# Autodesk Inventor assembly: Controller
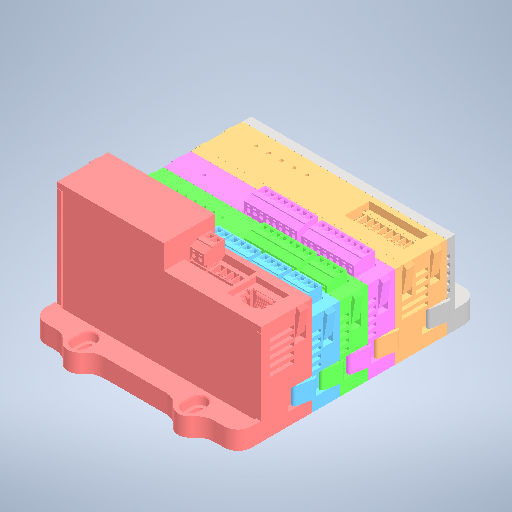
[picture p0: Inventor's stored thumbnail of the model, 512x512]
Saved by Autodesk Inventor 2025.2 (Build 292293000, 293)
## iProperties
Created: 2025-11-01
Part Number: Controller
Document SubType Name: Assembly
Designer: leowa
Author: leowa
## Documents named in this file (8)
- C:\Users\leowa\OneDrive - Fachhochschule Aachen\FH\8. Semester\CANTram-Framework\Inventor CAD\Workspaces\Arbeitsbereich\Module\Controller.iam
- C:\Users\leowa\OneDrive - Fachhochschule Aachen\FH\8. Semester\CANTram-Framework\Inventor CAD\Workspaces\Arbeitsbereich\Module\Analogmodul Baugruppe.iam
- C:\Users\leowa\OneDrive - Fachhochschule Aachen\FH\8. Semester\CANTram-Framework\Inventor CAD\Workspaces\Arbeitsbereich\Module\Busmodul Baugruppe.iam
- C:\Users\leowa\OneDrive - Fachhochschule Aachen\FH\8. Semester\CANTram-Framework\Inventor CAD\Workspaces\Arbeitsbereich\Module\Digitalmodul Baugruppe.iam
- C:\Users\leowa\OneDrive - Fachhochschule Aachen\FH\8. Semester\CANTram-Framework\Inventor CAD\Workspaces\Arbeitsbereich\Module\Hauptmodul.iam
- C:\Users\leowa\OneDrive - Fachhochschule Aachen\FH\8. Semester\CANTram-Framework\Inventor CAD\Workspaces\Arbeitsbereich\Gehäuse\Abschlussmodul.ipt
- C:\Users\leowa\OneDrive - Fachhochschule Aachen\FH\8. Semester\CANTram-Framework\Inventor CAD\Workspaces\Arbeitsbereich\Platinen\Debugmodul\Debugmodul\Debugmodul.iam
- C:\Users\leowa\OneDrive - Fachhochschule Aachen\FH\8. Semester\CANTram-Framework\Inventor CAD\Workspaces\Arbeitsbereich\Module\Relaismodul Baugruppe.iam
## Components (7 placed, 7 different names)
1. Analogmodul Baugruppe:1 [sub-assembly] — Fluchtend:1, Fluchtend:3, Fluchtend:4, Passend:1, Passend:2, Fluchtend:11
2. Busmodul Baugruppe:1 [sub-assembly] — Fluchtend:1, Fluchtend:2, Fluchtend:3, Passend:1, Fluchtend:5, Fluchtend:6, Fluchtend:9, Passend:5, Passend:6, Fluchtend:10, Passend:7
3. Digitalmodul Baugruppe:1 [sub-assembly] — Fluchtend:2, Fluchtend:4, Passend:2, Fluchtend:7, Fluchtend:8, Passend:4
4. Hauptmodul:1 [sub-assembly] — Fluchtend:7, Fluchtend:8, Passend:4
5. Abschlussmodul:1 — Fluchtend:5, Fluchtend:6, Passend:8
6. Debugmodul:1 [sub-assembly] — Fluchtend:9, Passend:5, Passend:6
7. Relaismodul Baugruppe:1 [sub-assembly] — Fluchtend:10, Fluchtend:11, Passend:7, Passend:8
## Relationships (18: Flush 11, Mate 7)
- Fluchtend:1 [Flush]: Analogmodul Baugruppe:1 ↔ Busmodul Baugruppe:1
- Fluchtend:2 [Flush]: Busmodul Baugruppe:1 ↔ Digitalmodul Baugruppe:1
- Fluchtend:3 [Flush]: Analogmodul Baugruppe:1 ↔ Busmodul Baugruppe:1
- Fluchtend:4 [Flush]: Analogmodul Baugruppe:1 ↔ Digitalmodul Baugruppe:1
- Passend:1 [Mate]: Analogmodul Baugruppe:1 ↔ Busmodul Baugruppe:1
- Passend:2 [Mate]: Analogmodul Baugruppe:1 ↔ Digitalmodul Baugruppe:1
- Fluchtend:5 [Flush]: Busmodul Baugruppe:1 ↔ Abschlussmodul:1
- Fluchtend:6 [Flush]: Busmodul Baugruppe:1 ↔ Abschlussmodul:1
- Fluchtend:7 [Flush]: Digitalmodul Baugruppe:1 ↔ Hauptmodul:1
- Fluchtend:8 [Flush]: Digitalmodul Baugruppe:1 ↔ Hauptmodul:1
- Passend:4 [Mate]: Digitalmodul Baugruppe:1 ↔ Hauptmodul:1
- Fluchtend:9 [Flush]: Busmodul Baugruppe:1 ↔ Debugmodul:1
- Passend:5 [Mate]: Busmodul Baugruppe:1 ↔ Debugmodul:1
- Passend:6 [Mate] (13.49 mm): Busmodul Baugruppe:1 ↔ Debugmodul:1
- Fluchtend:10 [Flush]: Busmodul Baugruppe:1 ↔ Relaismodul Baugruppe:1
- Fluchtend:11 [Flush]: Analogmodul Baugruppe:1 ↔ Relaismodul Baugruppe:1
- Passend:7 [Mate]: Busmodul Baugruppe:1 ↔ Relaismodul Baugruppe:1
- Passend:8 [Mate]: Abschlussmodul:1 ↔ Relaismodul Baugruppe:1
